# Autodesk Inventor assembly: left_arm
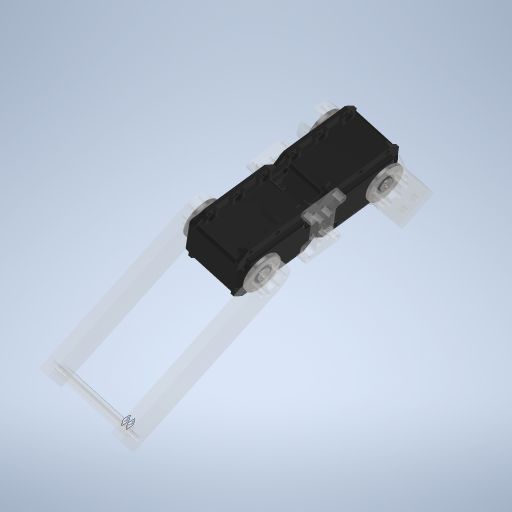
[picture p0: Inventor's stored thumbnail of the model, 512x512]
Saved by Autodesk Inventor 2024.3 (Build 283343000, 343)
## iProperties
Created: 2024-09-16
Part Number: left_arm
Document SubType Name: Assembly
Designer: USER
Author: USER
## Documents named in this file (7)
- C:\Users\USER\Desktop\로빛 예비인턴\(git)19기 이원준 격투로봇 설계파일\upper_body\left_arm.iam
- C:\Users\USER\Desktop\로빛 예비인턴\예비인턴 격투로봇 설계 프로젝트\격투로봇 백업 2\Motor_28.iam
- C:\Users\USER\Desktop\로빛 예비인턴\(git)19기 이원준 격투로봇 설계파일\upper_body\_arm_adt.ipt
- C:\Users\USER\Desktop\로빛 예비인턴\(git)19기 이원준 격투로봇 설계파일\upper_body\_hand_adt_ver_2_.ipt
- C:\Users\USER\Desktop\로빛 예비인턴\예비인턴 격투로봇 설계 프로젝트\_fist_ver2_.ipt
- C:\Users\USER\Desktop\로빛 예비인턴\(git)19기 이원준 격투로봇 설계파일\upper_body\_armpit_adt_1.ipt
- C:\Users\USER\Desktop\로빛 예비인턴\(git)19기 이원준 격투로봇 설계파일\upper_body\_arm_pti.ipt
## Components (10 placed, 6 different names)
1. Motor_28:1 [sub-assembly] — 각도:1
2. Motor_28:2 [sub-assembly] — 삽입:22
3. _arm_adt:1
4. _arm_adt:2
5. _hand_adt_ver_2_:1 — 삽입:22
6. _hand_adt_ver_2_:2 — 삽입:20, 삽입:21
7. _fist_ver2_:1 — 삽입:20, 삽입:21, 각도:2
8. _armpit_adt_1:1 — 각도:1, 각도:2
9. _armpit_adt_1:2
10. _arm_pti:1
## Relationships (22: Insert 18, Flush 2, Angle 2)
- [Insert]: _hand_adt_ver_2_:1 ↔ _fist_ver2_:1
- [Insert]: _hand_adt_ver_2_:1 ↔ _fist_ver2_:1
- [Insert]: Motor_28:2 ↔ _arm_adt:2
- [Insert]: Motor_28:2 ↔ _arm_adt:2
- [Insert]: Motor_28:1 ↔ _arm_adt:2
- [Insert]: Motor_28:1 ↔ _arm_adt:2
- [Insert]: Motor_28:1 ↔ _arm_adt:1
- [Insert]: Motor_28:2 ↔ _arm_adt:1
- [Insert]: Motor_28:2 ↔ _arm_adt:1
- [Insert]: Motor_28:1 ↔ _arm_adt:1
- [Flush]: _armpit_adt_1:2 ↔ _arm_pti:1
- [Flush]: _armpit_adt_1:2 ↔ _arm_pti:1
- [Insert]: _armpit_adt_1:1 ↔ _arm_pti:1
- [Insert]: _armpit_adt_1:1 ↔ _arm_pti:1
- [Insert]: _armpit_adt_1:2 ↔ _arm_pti:1
- [Insert]: _armpit_adt_1:2 ↔ _arm_pti:1
- [Insert]: Motor_28:1 ↔ _armpit_adt_1:2
- 각도:1 [Angle] (60 deg): Motor_28:1 ↔ _armpit_adt_1:1
- 삽입:20 [Insert]: _hand_adt_ver_2_:2 ↔ _fist_ver2_:1
- 삽입:21 [Insert]: _hand_adt_ver_2_:2 ↔ _fist_ver2_:1
- 각도:2 [Angle] (0 deg): _fist_ver2_:1 ↔ _armpit_adt_1:1
- 삽입:22 [Insert]: Motor_28:2 ↔ _hand_adt_ver_2_:1
## Named parameters: d18_d20 = 0 mm
